# Autodesk Inventor assembly: Assembly1
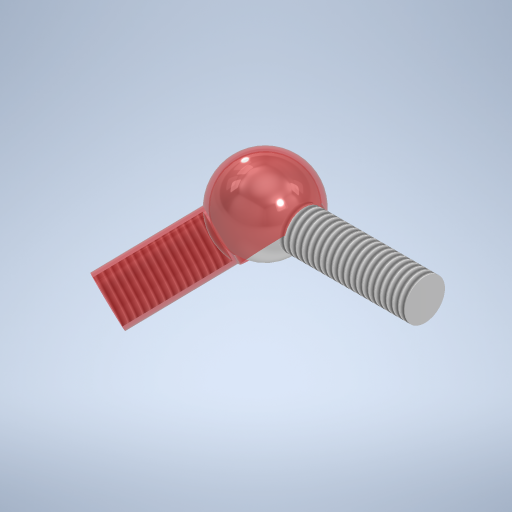
[picture p0: Inventor's stored thumbnail of the model, 512x512]
Saved by Autodesk Inventor 2023 (Build 270158000, 158)
## iProperties
Created: 2022-06-23
Part Number: Assembly1
Document SubType Name: Assembly
Designer: earls
Author: earls
## Documents named in this file (3)
- F:\Documents\Mechatronic Engineering 5.1\Project\CAD\Spherical joint\Assembly1.iam
- F:\Documents\Mechatronic Engineering 5.1\Project\CAD\Spherical joint\Part1.ipt
- F:\Documents\Mechatronic Engineering 5.1\Project\CAD\Spherical joint\Part2.ipt
## Components (2 placed, 2 different names)
1. Part1:1 — Ball:1
2. Part2:1 — Ball:1
## Relationships (1: BallJoint 1)
- Ball:1: Part1:1 ↔ Part2:1
